# Autodesk Inventor assembly: 組合1
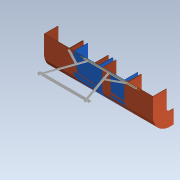
[picture p0: Inventor's stored thumbnail of the model, 180x180]
Saved by Autodesk Inventor 2022 (Build 260153000, 153)
## iProperties
Created: 2023-04-16
Part Number: 組合1
Document SubType Name: Assembly
Designer: JOU
Author: JOU
## Documents named in this file (6)
- C:\Users\Johnny Jou\Documents\GitHub\Areo_Rider_Cabin\test\組合1.iam
- C:\Users\Johnny Jou\Documents\GitHub\Areo_Rider_Cabin\test\零件1.ipt
- C:\Users\Johnny Jou\Documents\GitHub\Areo_Rider_Cabin\test\零件2.ipt
- C:\Users\Johnny Jou\Documents\GitHub\Areo_Rider_Cabin\test\零件3.ipt
- C:\Users\Johnny Jou\Documents\GitHub\Areo_Rider_Cabin\test\零件4.ipt
- C:\Users\Johnny Jou\Documents\GitHub\Areo_Rider_Cabin\Airfoil & Nuzzle\nuzzle\nuzzle_v2_0327.ipt
## Components (9 placed, 5 different names)
1. 零件1:1 — 插入:1, 插入:2, 角度:1
2. 零件2:1 — 插入:1, 插入:3, 貼合:2
3. 零件2:2 — 插入:2, 插入:4, 貼合:3
4. 零件3:1 — 插入:3, 貼合:1, 貼合:9
5. 零件3:2 — 插入:4, 貼合:4, 貼合:5, 貼合:8
6. 零件4:1 — 貼合:1, 貼合:2, 貼合:3, 貼合:4, 角度:1, 貼合:5, 貼合:6, 齊平:1
7. nuzzle_v2_0327:1 — 貼合:6, 齊平:1, 貼合:7, 齊平:2, 齊平:3, 齊平:4, 齊平:5
8. nuzzle_v2_0327:2 — 齊平:3, 齊平:4, 貼合:8
9. nuzzle_v2_0327:3 — 齊平:2, 齊平:5, 貼合:9
## Relationships (19: Mate 9, Flush 5, Insert 4, Angle 1)
- 插入:1 [Insert]: 零件1:1 ↔ 零件2:1
- 插入:2 [Insert]: 零件1:1 ↔ 零件2:2
- 插入:3 [Insert]: 零件2:1 ↔ 零件3:1
- 插入:4 [Insert]: 零件2:2 ↔ 零件3:2
- 貼合:1 [Mate]: 零件3:1 ↔ 零件4:1
- 貼合:2 [Mate]: 零件2:1 ↔ 零件4:1
- 貼合:3 [Mate]: 零件2:2 ↔ 零件4:1
- 貼合:4 [Mate]: 零件3:2 ↔ 零件4:1
- 角度:1 [Angle] (0 deg): 零件1:1 ↔ 零件4:1
- 貼合:5 [Mate]: 零件3:2 ↔ 零件4:1
- 貼合:6 [Mate]: 零件4:1 ↔ nuzzle_v2_0327:1
- 齊平:1 [Flush]: 零件4:1 ↔ nuzzle_v2_0327:1
- 貼合:7 [Mate] (5 mm): nuzzle_v2_0327:1
- 齊平:2 [Flush]: nuzzle_v2_0327:1 ↔ nuzzle_v2_0327:3
- 齊平:3 [Flush]: nuzzle_v2_0327:1 ↔ nuzzle_v2_0327:2
- 齊平:4 [Flush]: nuzzle_v2_0327:1 ↔ nuzzle_v2_0327:2
- 齊平:5 [Flush]: nuzzle_v2_0327:1 ↔ nuzzle_v2_0327:3
- 貼合:8 [Mate]: 零件3:2 ↔ nuzzle_v2_0327:2
- 貼合:9 [Mate]: 零件3:1 ↔ nuzzle_v2_0327:3
